# Autodesk Inventor assembly: Small Suction Cup 1764
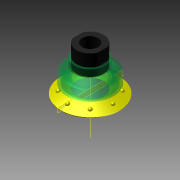
[picture p0: Inventor's stored thumbnail of the model, 180x180]
Saved by Autodesk Inventor 2011 (Build 150239000, 239)
## iProperties
Created: 2011-01-15
Part Number: Small Suction Cup 1764
Document SubType Name: Assembly
Designer: dfranz
Author: dfranz
## Documents named in this file (4)
- R:\CAD Archives\Pnewmatics\Suction Cups\Small Suction Cup 1764\Small Suction Cup 1764.iam
- R:\CAD Archives\Pnewmatics\Suction Cups\Small Suction Cup 1764\Small Suction Cup Part 1 1764.ipt
- R:\CAD Archives\Pnewmatics\Suction Cups\Small Suction Cup 1764\Small Suction Cup Part 2 1764.ipt
- R:\CAD Archives\Pnewmatics\Suction Cups\Small Suction Cup 1764\Small Suction Cup Part 3 1764.ipt
## Components (3 placed, 3 different names)
1. Small Suction Cup Part 1 1764:1 — Mate:1, Mate:2, Mate:3, Mate:4
2. Small Suction Cup Part 2 1764:1 — Mate:1, Mate:2
3. Small Suction Cup Part 3 1764:1 — Mate:3, Mate:4
## Relationships (4: Mate 4)
- Mate:1: Small Suction Cup Part 1 1764:1 ↔ Small Suction Cup Part 2 1764:1
- Mate:2: Small Suction Cup Part 1 1764:1 ↔ Small Suction Cup Part 2 1764:1
- Mate:3: Small Suction Cup Part 1 1764:1 ↔ Small Suction Cup Part 3 1764:1
- Mate:4: Small Suction Cup Part 1 1764:1 ↔ Small Suction Cup Part 3 1764:1
